# Autodesk Inventor assembly: breadplateConfig
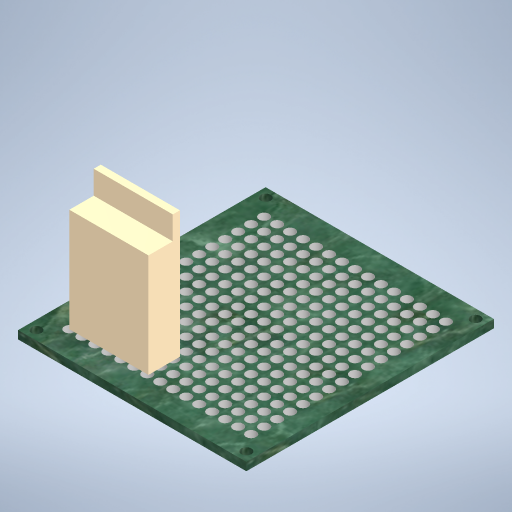
[picture p0: Inventor's stored thumbnail of the model, 512x512]
Saved by Autodesk Inventor 2023 (Build 270158000, 158)
## iProperties
Created: 2023-09-27
Part Number: breadplateConfig
Document SubType Name: Assembly
Designer: Gage
Author: Gage
## Documents named in this file (3)
- C:\Users\Gage\OneDrive\Desktop\Autodesk Inventor\breadplateConfig.iam
- C:\Users\Gage\OneDrive\Desktop\Autodesk Inventor\breadplate.ipt
- C:\Users\Gage\OneDrive\Desktop\Autodesk Inventor\DHT22.ipt
## Components (2 placed, 2 different names)
1. breadplate:1 — Mate:1, Mate:2, Mate:3
2. DHT22:1 — Mate:1, Mate:2, Mate:3
## Relationships (3: Mate 3)
- Mate:1: breadplate:1 ↔ DHT22:1
- Mate:2: breadplate:1 ↔ DHT22:1
- Mate:3: breadplate:1 ↔ DHT22:1
